# Autodesk Inventor assembly: IRB120
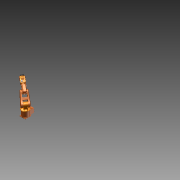
[picture p0: Inventor's stored thumbnail of the model, 180x180]
Saved by Autodesk Inventor 2012 (Build 160160000, 160)
## iProperties
Created: 2011-12-25
Part Number: IRB120
Document SubType Name: Assembly
Designer: Ed
Mass: 18023.2 g
Surface Area: 14043.7 cm^2
Volume: 18023.2 cm^3
Density: 1 g/cm^3
Translation Standard: STEP AP214IS
FileName: IRB120_3-58_IRC5_rev0.STEP
PreProcessor: SolidWorks 2008
PostProcessor: Build: 160, Release: 2012 RTM - Date: Tue 03/01/2011
Sent Units: millimeter
Uncertainty: 1e-05
Author: Ed
## Documents named in this file (8)
- C:\Users\Ed\armbot\IRB120\IRB120.iam
- C:\Users\Ed\armbot\IRB120\Inventor Parts\IRB120_Link6_rev0.ipt
- C:\Users\Ed\armbot\IRB120\Inventor Parts\IRB120_Link3_rev0.iam
- C:\Users\Ed\armbot\IRB120\Inventor Parts\IRB120_Link1_rev0.iam
- C:\Users\Ed\armbot\IRB120\Inventor Parts\IRB120_Base_rev0.iam
- C:\Users\Ed\armbot\IRB120\Inventor Parts\IRB120_Link2_rev0.iam
- C:\Users\Ed\armbot\IRB120\Inventor Parts\IRB120_Link4_rev0.iam
- C:\Users\Ed\armbot\IRB120\Inventor Parts\IRB120_Link5_rev0.iam
## Components (7 placed, 7 different names)
1. IRB120_Link6_rev0:1 — Mate:6, Flush:1
2. IRB120_Link3_rev0:1 [sub-assembly] — Mate:3, Mate:4, Mate:7, Mate:8
3. IRB120_Link1_rev0:1 [sub-assembly] — Mate:1, Mate:2, Mate:9, Mate:10
4. IRB120_Base_rev0:1 [sub-assembly] — Mate:2, Mate:10
5. IRB120_Link2_rev0:1 [sub-assembly] — Mate:1, Mate:3, Mate:8, Mate:9
6. IRB120_Link4_rev0:1 [sub-assembly] — Mate:4, Mate:5, Mate:7, Mate:11
7. IRB120_Link5_rev0:1 [sub-assembly] — Mate:5, Mate:6, Flush:1, Mate:11
## Relationships (12: Mate 11, Flush 1)
- Mate:1: IRB120_Link1_rev0:1 ↔ IRB120_Link2_rev0:1
- Mate:2: IRB120_Link1_rev0:1 ↔ IRB120_Base_rev0:1
- Mate:3: IRB120_Link3_rev0:1 ↔ IRB120_Link2_rev0:1
- Mate:4: IRB120_Link3_rev0:1 ↔ IRB120_Link4_rev0:1
- Mate:5: IRB120_Link4_rev0:1 ↔ IRB120_Link5_rev0:1
- Mate:6: IRB120_Link6_rev0:1 ↔ IRB120_Link5_rev0:1
- Flush:1 (-6.5 mm): IRB120_Link6_rev0:1 ↔ IRB120_Link5_rev0:1
- Mate:7 (6.4 mm): IRB120_Link3_rev0:1 ↔ IRB120_Link4_rev0:1
- Mate:8 (9 mm): IRB120_Link3_rev0:1 ↔ IRB120_Link2_rev0:1
- Mate:9 (7.5 mm): IRB120_Link1_rev0:1 ↔ IRB120_Link2_rev0:1
- Mate:10 (2 mm): IRB120_Link1_rev0:1 ↔ IRB120_Base_rev0:1
- Mate:11 (1 mm): IRB120_Link4_rev0:1 ↔ IRB120_Link5_rev0:1
